# Autodesk Inventor assembly: GP-56012
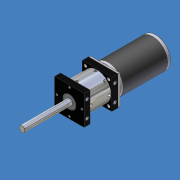
[picture p0: Inventor's stored thumbnail of the model, 180x180]
Saved by Autodesk Inventor 2012 (Build 160160000, 160)
## iProperties
Company: First Team 34
Shininess: 64.0
Length Units: 11269
Angle Units: 11279
Time Units: 11290
Mass Units: 11283
Length Display Precision: 3
Angle Display Precision: 2
Compacted: True
Created: 2007-01-08
Part Number: GP-56012
Document SubType Name: Assembly
Designer: Ed Sparks
Catalog Web Link: www.banebots.com
Vendor: BaneBots
Description: BaneBots GP-56012 Gearbox 12:1
Mass: 1788.53 g
Surface Area: 1044.7 cm^2
Volume: 533.915 cm^3
Density: 3.34983 g/cm^3
Density: 0.0
Volumn: 0.0
Area: 0.0
PropertySet Name: Model Information
Control State: 0
Master: False
Checked Out: False
Title: BaneBot GP-56012
Subject: BaneBot
Author: Ed Sparks
## Documents named in this file (8)
- C:\Users\Andrew G. Meyer\Documents\Projects\BallBot\macro\CAD\P80\BB-56012.iam
- C:\Users\Andrew G. Meyer\Documents\Projects\BallBot\macro\CAD\P80\BB2-InterfacePlate.ipt
- C:\Users\Andrew G. Meyer\Documents\Projects\BallBot\macro\CAD\P80\BB2-BackPlate.ipt
- C:\Users\Andrew G. Meyer\Documents\Projects\BallBot\macro\CAD\P80\BB2-RingGear.ipt
- C:\Users\Andrew G. Meyer\Documents\Projects\BallBot\macro\CAD\P80\BB2-FrontPlate.ipt
- C:\Users\Andrew G. Meyer\Documents\Projects\BallBot\macro\CAD\P80\br-8.ipt
- C:\Users\Andrew G. Meyer\Documents\Projects\BallBot\macro\CAD\P80\BB2-OutputShaft.ipt
- C:\Users\Andrew G. Meyer\Documents\Projects\BallBot\macro\CAD\P80\CIM Motor.iam
## Components (8 placed, 7 different names)
1. BB2-InterfacePlate:1 — Mate:1, Angle:1, Mate:2, Mate:14, Mate:15
2. BB2-BackPlate:1 — Mate:1, Angle:1, Mate:2, Mate:3, Mate:4, Mate:5, Angle:2
3. BB2-RingGear:1 — Mate:3, Mate:4, Mate:5, Mate:6, Mate:7
4. BB2-FrontPlate:1 — Mate:6, Mate:7, Mate:10, Flush:1, Angle:2
5. br-8:1 — Mate:8, Mate:9, Mate:10, Flush:1, Mate:11, Mate:12
6. br-8:2 — Mate:8, Mate:9
7. BB2-OutputShaft:1 — Mate:11, Mate:12, Mate:13
8. CIM Motor:1 [sub-assembly] — Mate:13, Mate:14, Mate:15
## Relationships (18: Mate 15, Angle 2, Flush 1)
- Mate:1: BB2-InterfacePlate:1 ↔ BB2-BackPlate:1
- Angle:1 (0 deg): BB2-InterfacePlate:1 ↔ BB2-BackPlate:1
- Mate:2: BB2-InterfacePlate:1 ↔ BB2-BackPlate:1
- Mate:3: BB2-BackPlate:1 ↔ BB2-RingGear:1
- Mate:4: BB2-BackPlate:1 ↔ BB2-RingGear:1
- Mate:5: BB2-BackPlate:1 ↔ BB2-RingGear:1
- Mate:6: BB2-RingGear:1 ↔ BB2-FrontPlate:1
- Mate:7: BB2-RingGear:1 ↔ BB2-FrontPlate:1
- Mate:8: br-8:1 ↔ br-8:2
- Mate:9: br-8:1 ↔ br-8:2
- Mate:10: BB2-FrontPlate:1 ↔ br-8:1
- Flush:1: BB2-FrontPlate:1 ↔ br-8:1
- Mate:11: br-8:1 ↔ BB2-OutputShaft:1
- Mate:12 (-101.6 mm): br-8:1 ↔ BB2-OutputShaft:1
- Angle:2 (0 deg): BB2-BackPlate:1 ↔ BB2-FrontPlate:1
- Mate:13: BB2-OutputShaft:1 ↔ CIM Motor:1
- Mate:14: BB2-InterfacePlate:1 ↔ CIM Motor:1
- Mate:15: BB2-InterfacePlate:1 ↔ CIM Motor:1
